# Autodesk Inventor assembly: Motor-Bracket-with-inserts
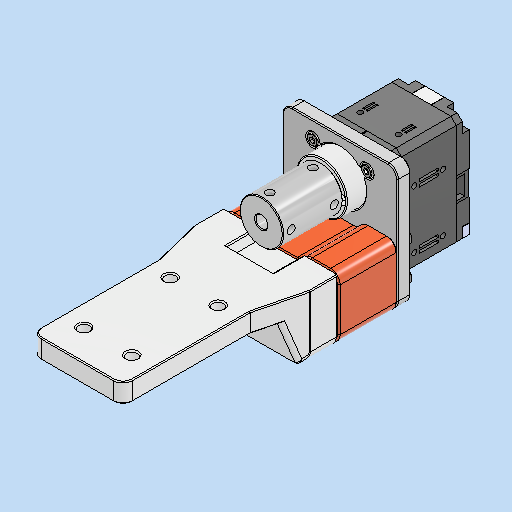
[picture p0: Inventor's stored thumbnail of the model, 512x512]
Saved by Autodesk Inventor 2025 (Build 290162000, 162)
## iProperties
Created: 2025-05-29
Part Number: Motor-Bracket-with-inserts
Document SubType Name: Assembly
Designer: kuzmin
Mass: 45.0024 g
Surface Area: 124.627 cm^2
Volume: 41.0459 cm^3
Density: 1.09639 g/cm^3
Author: kuzmin
## Documents named in this file (9)
- C:\Users\queezz\Dropbox\Drawings\PIHTI\LIBS\Motor-Bracket-with-inserts.iam
- C:\Users\queezz\Dropbox\Drawings\PIHTI\LIBS\XL430_W250_T\XL430_W250_T.iam
- C:\Users\queezz\Dropbox\Drawings\PIHTI\LIBS\Motor-Plate.ipt
- C:\Users\queezz\Dropbox\Drawings\PIHTI\ContentCenter\Fastners\M2.5x10-SHCS.ipt
- C:\Users\queezz\Dropbox\Drawings\PIHTI\LIBS\Motor-Bracket-threaded.iam
- C:\Users\queezz\Dropbox\Drawings\PIHTI\LIBS\Motor-Bracket-spacer.ipt
- C:\Users\queezz\Dropbox\Drawings\PIHTI\LIBS\new-coupler.ipt
- C:\Users\queezz\Dropbox\Drawings\PIHTI\LIBS\spring-shaft-coupler.ipt
- C:\Users\queezz\Dropbox\Drawings\PIHTI\ContentCenter\Fastners\M3x35-SHCS.ipt
## Components (14 placed, 8 different names)
1. XL430_W250_T:1 [sub-assembly] — Flush:1, Rotational:1, Rotational:2, Mate:7
2. Motor-Plate:1 — Rigid:12, Rigid:13, Rigid:14, Rigid:15, Mate:4, Rotational:2, Flush:3, Flush:4, Mate:8, Rigid:17, Rigid:18, Rigid:19, Rigid:20
3. Motor-Bracket-threaded:1 [sub-assembly] — Mate:4, Mate:9
4. new-coupler:1 — Rotational:1, Mate:7, Rigid:16
5. spring-shaft-coupler:1 — Rigid:16
6. Motor-Bracket-spacer:1 — Flush:3, Flush:4, Mate:8, Mate:9
7. Unbrako Hex Socket Cap - Metric M3 x 35:1 — Rigid:20
8. Unbrako Hex Socket Cap - Metric M3 x 35:2 — Rigid:19
9. Unbrako Hex Socket Cap - Metric M3 x 35:3 — Rigid:18
10. Unbrako Hex Socket Cap - Metric M3 x 35:4 — Rigid:17
11. BS EN ISO 4762 - Metric M2,5 x 10:1 — Rigid:14
12. BS EN ISO 4762 - Metric M2,5 x 10:2 — Rigid:15
13. BS EN ISO 4762 - Metric M2,5 x 10:3 — Rigid:13
14. BS EN ISO 4762 - Metric M2,5 x 10:4 — Rigid:12
## Relationships (19: WeldJoint 9, Flush 4, Mate 4, RevoluteJoint 2)
- Flush:1: XL430_W250_T:1
- [Flush]: Motor-Bracket-threaded:1
- Rigid:12 [WeldJoint] (0.6 mm): Motor-Plate:1 ↔ BS EN ISO 4762 - Metric M2,5 x 10:4
- Rigid:13 [WeldJoint] (0.6 mm): Motor-Plate:1 ↔ BS EN ISO 4762 - Metric M2,5 x 10:3
- Rigid:14 [WeldJoint] (0.3 mm): Motor-Plate:1 ↔ BS EN ISO 4762 - Metric M2,5 x 10:1
- Rigid:15 [WeldJoint] (0.6 mm): Motor-Plate:1 ↔ BS EN ISO 4762 - Metric M2,5 x 10:2
- Mate:4: Motor-Plate:1 ↔ Motor-Bracket-threaded:1
- Rotational:1 [RevoluteJoint]: XL430_W250_T:1 ↔ new-coupler:1
- Rotational:2 [RevoluteJoint]: XL430_W250_T:1 ↔ Motor-Plate:1
- Mate:7: XL430_W250_T:1 ↔ new-coupler:1
- Rigid:16 [WeldJoint]: new-coupler:1 ↔ spring-shaft-coupler:1
- Flush:3: Motor-Plate:1 ↔ Motor-Bracket-spacer:1
- Flush:4: Motor-Plate:1 ↔ Motor-Bracket-spacer:1
- Mate:8: Motor-Plate:1 ↔ Motor-Bracket-spacer:1
- Mate:9: Motor-Bracket-threaded:1 ↔ Motor-Bracket-spacer:1
- Rigid:17 [WeldJoint]: Motor-Plate:1 ↔ Unbrako Hex Socket Cap - Metric M3 x 35:4
- Rigid:18 [WeldJoint]: Motor-Plate:1 ↔ Unbrako Hex Socket Cap - Metric M3 x 35:3
- Rigid:19 [WeldJoint]: Motor-Plate:1 ↔ Unbrako Hex Socket Cap - Metric M3 x 35:2
- Rigid:20 [WeldJoint]: Motor-Plate:1 ↔ Unbrako Hex Socket Cap - Metric M3 x 35:1
